# Autodesk Inventor assembly: Băng chuyền
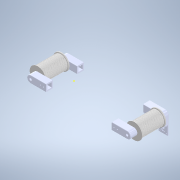
[picture p0: Inventor's stored thumbnail of the model, 180x180]
Saved by Autodesk Inventor 2020 (Build 240168000, 168)
## iProperties
Created: 2022-03-31
Part Number: Băng chuyền
Document SubType Name: Assembly
Designer: PC
Author: PC
## Documents named in this file (6)
- D:\Do-an-tot-nghiep\Băng chuyền.iam
- D:\Inventor 2020\bangchuyen\bangchuyen.ipt
- D:\Do-an-tot-nghiep\bangchuyenstep.ipt
- D:\Do-an-tot-nghiep\truc_bang_chuyen.ipt
- D:\Do-an-tot-nghiep\Trục băng chuyền.ipt
- D:\Do-an-tot-nghiep\Băng chuyền step.ipt
## Components (8 placed, 5 different names)
1. bangchuyen:1 — Flush:1, Flush:2, Flush:3, Mate:5, Mate:9
2. bangchuyenstep:1 — Mate:3, Mate:4, Flush:1, Flush:2, Flush:5
3. truc_bang_chuyen:1
4. Trục băng chuyền:1 — Mate:3, Mate:4, Mate:7
5. Băng chuyền step:1
6. bangchuyen:2 — Flush:3, Mate:5, Flush:4, Mate:6, Mate:8
7. bangchuyen:3 — Flush:4, Mate:6, Mate:7, Flush:5
8. Trục băng chuyền:2 — Mate:8, Mate:9
## Relationships (12: Mate 7, Flush 5)
- Mate:3: bangchuyenstep:1 ↔ Trục băng chuyền:1
- Mate:4: bangchuyenstep:1 ↔ Trục băng chuyền:1
- Flush:1: bangchuyen:1 ↔ bangchuyenstep:1
- Flush:2: bangchuyen:1 ↔ bangchuyenstep:1
- Flush:3: bangchuyen:1 ↔ bangchuyen:2
- Mate:5: bangchuyen:1 ↔ bangchuyen:2
- Flush:4: bangchuyen:2 ↔ bangchuyen:3
- Mate:6: bangchuyen:2 ↔ bangchuyen:3
- Mate:7: Trục băng chuyền:1 ↔ bangchuyen:3
- Flush:5: bangchuyenstep:1 ↔ bangchuyen:3
- Mate:8: bangchuyen:2 ↔ Trục băng chuyền:2
- Mate:9: bangchuyen:1 ↔ Trục băng chuyền:2
